# Autodesk Inventor assembly: Elevator Motor Assembly
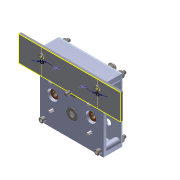
[picture p0: Inventor's stored thumbnail of the model, 180x180]
Saved by Autodesk Inventor 2015 (Build 190159000, 159)
## iProperties
Created: 2015-01-24
Part Number: Elevator Motor Assembly
Document SubType Name: Assembly
Designer: Peter
Author: Peter
## Documents named in this file (3)
- T:\FILES\FIRST-Team-1719-CAD-Team\2015 Robot CAD\Two Lifters and Lifter Super Structure\Lifter Super Structure\Tower\Elevator Motor Assembly\Elevator Motor Assembly.iam
- T:\FILES\FIRST-Team-1719-CAD-Team\2015 Robot CAD\Two Lifters and Lifter Super Structure\Lifter Super Structure\Tower\Elevator Motor Assembly\Lower Motor Mount.ipt
- T:\FILES\FIRST-Team-1719-CAD-Team\2015 Robot CAD\Two Lifters and Lifter Super Structure\Lifter Super Structure\Tower\Elevator Motor Assembly\Andy Mark Tough Box.iam
## Components (2 placed, 2 different names)
1. Lower Motor Mount:1 — Mate:1, Flush:1
2. Andy Mark Tough Box:1 [sub-assembly] — Mate:1, Flush:1
## Relationships (2: Mate 1, Flush 1)
- Mate:1: Lower Motor Mount:1 ↔ Andy Mark Tough Box:1
- Flush:1 (38.1 mm): Lower Motor Mount:1 ↔ Andy Mark Tough Box:1
